# Autodesk Inventor assembly: Camera Assembly
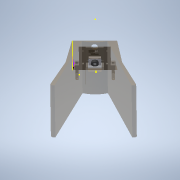
[picture p0: Inventor's stored thumbnail of the model, 180x180]
Saved by Autodesk Inventor 2022 (Build 260153000, 153)
## iProperties
Created: 2023-03-07
Part Number: Camera Assembly
Document SubType Name: Assembly
Designer: zarek
Author: zarek
## Documents named in this file (3)
- C:\Users\zarek\OneDrive\Desktop\Random New Stuff\SPB\Camera Assembly.iam
- C:\Users\zarek\OneDrive\Desktop\Random New Stuff\SPB\Camera_Holder - Copy.ipt
- C:\Users\zarek\OneDrive\Desktop\Random New Stuff\SPB\Camera & Angle.iam
## Components (2 placed, 2 different names)
1. Camera_Holder - Copy:1 — Rotational:1
2. Camera & Angle:1 [sub-assembly] — Rotational:1
## Relationships (1: RevoluteJoint 1)
- Rotational:1 [RevoluteJoint]: Camera_Holder - Copy:1 ↔ Camera & Angle:1
